# Autodesk Inventor assembly: 000-A-000
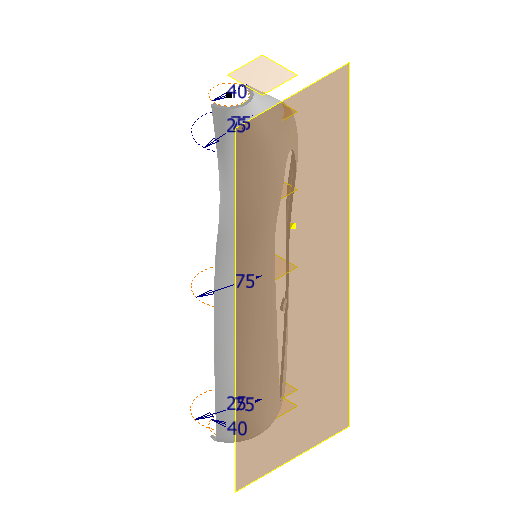
[picture p0: Inventor's stored thumbnail of the model, 512x512]
Saved by Autodesk Inventor 2025.1 (Build 291241000, 241)
## iProperties
Created: 2025-01-27
Part Number: 000-A-000
Document SubType Name: Assembly
Designer: alptl
Category: <PROJECT CATAGORY>
Title: <TITLE>
Author: alptl
Revision Number: A
## Documents named in this file (3)
- C:\Users\alptl\Desktop\fairingfghj.iam
- C:\Users\alptl\Desktop\fairibg.ipt
- C:\Users\me19654\OneDrive - University of Bristol\PhD Project\005 Design (CAD and schematics)\001 Wind Tunnel\CAD Library\001-A-017 CONTRACTION ASSY.iam
## Components (1 placed, 1 different names)
1. fairibg:1 — Flush:1
## Relationships (1: Flush 1)
- Flush:1: fairibg:1
